# Autodesk Inventor assembly: v2RevA
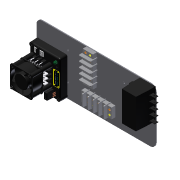
[picture p0: Inventor's stored thumbnail of the model, 180x180]
Saved by Autodesk Inventor 2015 (Build 190159000, 159)
## iProperties
Created: 2013-12-30
Part Number: v2RevA
Document SubType Name: Assembly
Designer: davidgitz
Author: davidgitz
## Documents named in this file (6)
- C:\SharedDrive\Dropbox\ICARUS\Rover\MECHANICAL\810002_ASY-FAST ROVER v2\813006_FAST ROVER v2 CHASSIS ELECTRONICS\813006_FAST ROVER v2 CHASSIS ELECTRONICS.iam
- C:\SharedDrive\Dropbox\ICARUS\Rover\MECHANICAL\810002_ASY-FAST ROVER v2\813006_FAST ROVER v2 CHASSIS ELECTRONICS\Hex Offset.ipt
- C:\SharedDrive\Dropbox\ICARUS\Rover\MECHANICAL\810002_ASY-FAST ROVER v2\813006_FAST ROVER v2 CHASSIS ELECTRONICS\Plate.ipt
- C:\SharedDrive\Dropbox\ICARUS\Rover\MECHANICAL\810002_ASY-FAST ROVER v2\813006_FAST ROVER v2 CHASSIS ELECTRONICS\362000_Victor 884 Motor Controller\362000_Victor 884 Motor Controller.iam
- C:\SharedDrive\Dropbox\ICARUS\Rover\MECHANICAL\810002_ASY-FAST ROVER v2\813006_FAST ROVER v2 CHASSIS ELECTRONICS\FuseBlock.ipt
- C:\SharedDrive\Dropbox\ICARUS\Rover\MECHANICAL\810002_ASY-FAST ROVER v2\813006_FAST ROVER v2 CHASSIS ELECTRONICS\Terminal Block.ipt
## Components (9 placed, 6 different names)
1. Hex Offset:1 — Insert:41
2. Plate:1 — Mate:16, Flush:13, Flush:14, Insert:41, Insert:42, Insert:43, Insert:44, Mate:66, Mate:72, Mate:73, Flush:31, Mate:74, Mate:75, Mate:76, Mate:77, Flush:32, Angle:1
3. 362000_Victor 884 Motor Controller:1 [sub-assembly] — Mate:75, Mate:76, Mate:77
4. FuseBlock:1 — Mate:16, Flush:13, Flush:14
5. 6V PDB — Mate:66, Flush:32
6. Hex Offset:2 — Insert:42
7. Hex Offset:3 — Insert:43
8. Hex Offset:4 — Insert:44
9. Terminal Block:3 — Mate:74, Angle:1
## Relationships (17: Mate 8, Flush 4, Insert 4, Angle 1)
- Mate:16: Plate:1 ↔ FuseBlock:1
- Flush:13: Plate:1 ↔ FuseBlock:1
- Flush:14: Plate:1 ↔ FuseBlock:1
- Insert:41: Hex Offset:1 ↔ Plate:1
- Insert:42: Plate:1 ↔ Hex Offset:2
- Insert:43: Plate:1 ↔ Hex Offset:3
- Insert:44: Plate:1 ↔ Hex Offset:4
- Mate:66: Plate:1 ↔ 6V PDB
- Mate:72: Plate:1
- Mate:73: Plate:1
- Flush:31: Plate:1
- Mate:74: Plate:1 ↔ Terminal Block:3
- Mate:75: Plate:1 ↔ 362000_Victor 884 Motor Controller:1
- Mate:76: Plate:1 ↔ 362000_Victor 884 Motor Controller:1
- Mate:77: Plate:1 ↔ 362000_Victor 884 Motor Controller:1
- Flush:32: Plate:1 ↔ 6V PDB
- Angle:1 (0 deg): Plate:1 ↔ Terminal Block:3
